# Autodesk Inventor assembly: Ensamblaje 1 Carlos Lucero No.1184321
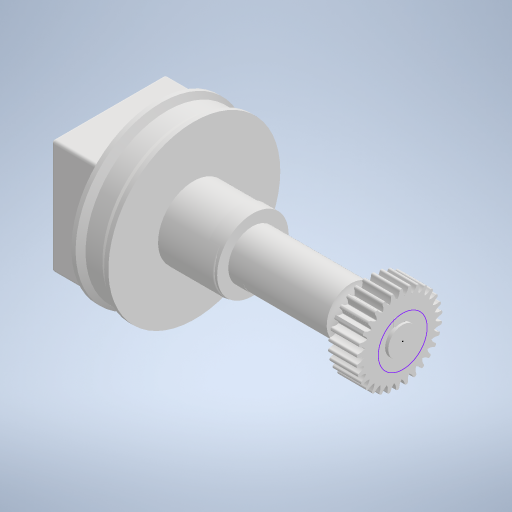
[picture p0: Inventor's stored thumbnail of the model, 512x512]
Saved by Autodesk Inventor 2024 (Build 280153000, 153)
## iProperties
Created: 2024-03-31
Part Number: Ensamblaje 1 Carlos Lucero No.1184321
Document SubType Name: Assembly
Designer: Andres
Author: Andres
## Documents named in this file (7)
- C:\Users\Andres\OneDrive\Escritorio\U\Primer Semestre año 2024\Lab Dinamica\Ensamblaje 1 Carlos Lucero No.1184321.iam
- C:\Users\Andres\OneDrive\Escritorio\U\Primer Semestre año 2024\Lab Dinamica\POLEA.ipt
- C:\Users\Andres\OneDrive\Escritorio\U\Primer Semestre año 2024\Lab Dinamica\EJE_CUÑEROS.ipt
- C:\Users\Andres\OneDrive\Escritorio\U\Primer Semestre año 2024\Lab Dinamica\CUÑA.ipt
- C:\Users\Andres\OneDrive\Escritorio\U\Primer Semestre año 2024\Lab Dinamica\ENGRANE.ipt
- C:\Users\Andres\OneDrive\Escritorio\U\Primer Semestre año 2024\Lab Dinamica\PRACTICA #1 CONOCIENDO INVENTOR CARLOS LUCERO NO. 1184321.ipt
- C:\Users\Andres\OneDrive\Escritorio\U\Primer Semestre año 2024\Lab Dinamica\piezaaa.ipt
## Components (7 placed, 6 different names)
1. EJE_CUÑEROS:1 — Rígido:1, Rígido:2, Rígido:3, Cilíndrica:1, Coincidencia:1
2. ENGRANE:1 — Cilíndrica:1
3. POLEA:1 — Rígido:3
4. CUÑA:2 — Rígido:1
5. CUÑA:3 — Rígido:2
6. PRACTICA #1 CONOCIENDO INVENTOR CARLOS LUCERO NO. 1184321:1 — Coincidencia:1
7. piezaaa:1
## Relationships (5: WeldJoint 3, CylindricalJoint 1, Mate 1)
- Rígido:1 [WeldJoint]: EJE_CUÑEROS:1 ↔ CUÑA:2
- Rígido:2 [WeldJoint]: EJE_CUÑEROS:1 ↔ CUÑA:3
- Rígido:3 [WeldJoint]: EJE_CUÑEROS:1 ↔ POLEA:1
- Cilíndrica:1 [CylindricalJoint]: EJE_CUÑEROS:1 ↔ ENGRANE:1
- Coincidencia:1 [Mate]: EJE_CUÑEROS:1 ↔ PRACTICA #1 CONOCIENDO INVENTOR CARLOS LUCERO NO. 1184321:1
